# Autodesk Inventor assembly: Darrieus Turbine Assy
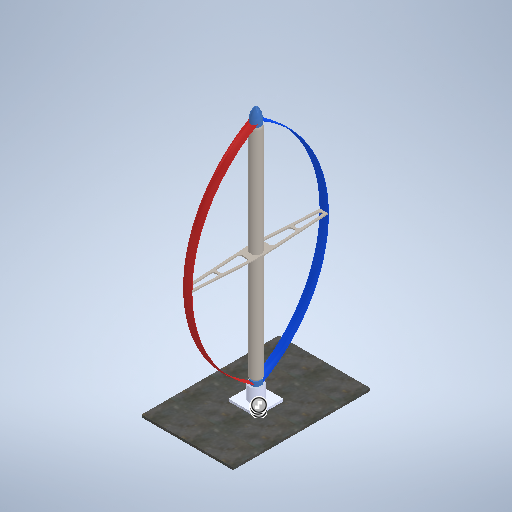
[picture p0: Inventor's stored thumbnail of the model, 512x512]
Saved by Autodesk Inventor 2025.4 (Build 294407000, 407)
## iProperties
Created: 2012-03-26
Part Number: Darrieus Turbine Assy
Description: STEP AP214
Document SubType Name: Assembly
Designer: Mathieu
Sending System: SolidWorks 2012
Preprocessor: SwSTEP 2.0
Title: Darrieus Turbine Assy.STEP
Author: 4745G
Revision Number: ANY
## Documents named in this file (8)
- C:\Users\louis\OneDrive\Desktop\R_Trident\02_CAD\08_Template\VisAssemblage-Tutoriel-FixationEolienne\Darrieus Turbine Assy.iam
- C:\Users\louis\OneDrive\Desktop\R_Trident\02_CAD\08_Template\VisAssemblage-Tutoriel-FixationEolienne\Mat.ipt
- C:\Users\louis\OneDrive\Desktop\R_Trident\02_CAD\08_Template\VisAssemblage-Tutoriel-FixationEolienne\Airfoil Darieus NACA 63-212.ipt
- C:\Users\louis\OneDrive\Desktop\R_Trident\02_CAD\08_Template\VisAssemblage-Tutoriel-FixationEolienne\Pied.ipt
- C:\Users\louis\OneDrive\Desktop\R_Trident\02_CAD\08_Template\VisAssemblage-Tutoriel-FixationEolienne\PlaqueSupport.ipt
- C:\Users\louis\OneDrive\Documents\Inventor\Content Center Files\R2025\en-US\ISO 4762(2)\ISO 4762 - M8 x 30ISO.ipt
- C:\Users\louis\OneDrive\Documents\Inventor\Content Center Files\R2025\en-US\ISO 7092\ISO 7092 - ST 8 - 140 HV.ipt
- C:\Users\louis\OneDrive\Documents\Inventor\Content Center Files\R2025\en-US\ISO 4035(2)\ISO 4035 - M8 - ISO.ipt
## Components (7 placed, 7 different names)
1. Pied — Mate:1, Mate:2, Mate:3, Mate:4, Mate:5, Mate:8, Mate:9, Mate:10
2. Mat — Mate:6, Mate:7
3. Airfoil Darieus NACA 63-212_2 — Mate:4, Mate:5, Mate:6, Mate:7
4. PlaqueSupport:1 — Mate:1, Mate:2, Mate:3, Mate:11
5. ISO 4762 M8 x 30:1 — Mate:8, Mate:9
6. ISO 7092 ST 8 - 140 HV:1 — Mate:10, Mate:11, Insert:1
7. ISO 4035 M8:1 — Insert:1
## Relationships (12: Mate 11, Insert 1)
- Mate:1: Pied ↔ PlaqueSupport:1
- Mate:2: Pied ↔ PlaqueSupport:1
- Mate:3: Pied ↔ PlaqueSupport:1
- Mate:4: Pied ↔ Airfoil Darieus NACA 63-212_2
- Mate:5: Pied ↔ Airfoil Darieus NACA 63-212_2
- Mate:6: Mat ↔ Airfoil Darieus NACA 63-212_2
- Mate:7: Mat ↔ Airfoil Darieus NACA 63-212_2
- Mate:8: Pied ↔ ISO 4762 M8 x 30:1
- Mate:9: Pied ↔ ISO 4762 M8 x 30:1
- Mate:10: Pied ↔ ISO 7092 ST 8 - 140 HV:1
- Mate:11: PlaqueSupport:1 ↔ ISO 7092 ST 8 - 140 HV:1
- Insert:1: ISO 7092 ST 8 - 140 HV:1 ↔ ISO 4035 M8:1
